# Autodesk Inventor assembly: Montagem1
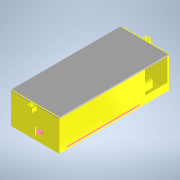
[picture p0: Inventor's stored thumbnail of the model, 180x180]
Saved by Autodesk Inventor 2022 (Build 260153000, 153)
## iProperties
Created: 2024-03-03
Part Number: Montagem1
Document SubType Name: Assembly
Designer: Daniel
Author: Daniel
## Documents named in this file (4)
- C:\Users\Daniel\Documents\Inventor\prototipoV4\Montagem1.iam
- C:\Users\Daniel\Documents\Inventor\prototipoV4\ArduinoMega_STEP_AP203.ipt
- C:\Users\Daniel\Documents\Inventor\prototipoV4\basecaixa.ipt
- C:\Users\Daniel\Documents\Inventor\prototipoV4\tampa.ipt
## Components (3 placed, 3 different names)
1. ArduinoMega_STEP_AP203:1 — Coincidente:1
2. basecaixa:1 — Coincidente:1, Alinhado:1, Coincidente:2, Alinhado:2
3. tampa:1 — Alinhado:1, Coincidente:2, Alinhado:2
## Relationships (4: Mate 2, Flush 2)
- Coincidente:1 [Mate]: ArduinoMega_STEP_AP203:1 ↔ basecaixa:1
- Alinhado:1 [Flush]: basecaixa:1 ↔ tampa:1
- Coincidente:2 [Mate]: basecaixa:1 ↔ tampa:1
- Alinhado:2 [Flush]: basecaixa:1 ↔ tampa:1
